# Autodesk Inventor assembly: Sosna
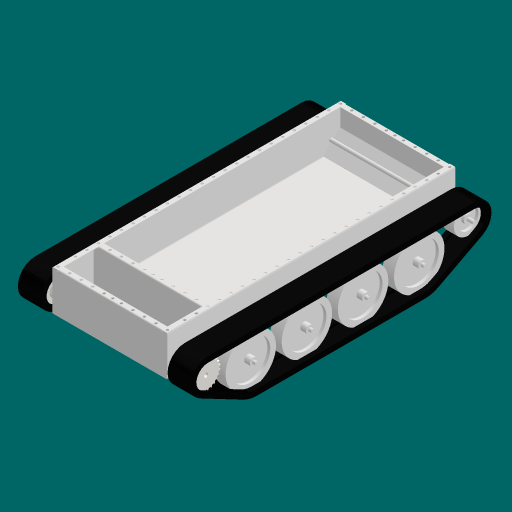
[picture p0: Inventor's stored thumbnail of the model, 512x512]
Saved by Autodesk Inventor 2023 (Build 270158000, 158)
## iProperties
Created: 2023-01-04
Part Number: Sosna
Document SubType Name: Weldment
Designer: HeavyDrewno
Weld Material: Welded Aluminum-6061
Author: HeavyDrewno
## Documents named in this file (16)
- C:\Users\HeavyDrewno\Desktop\Sosna\Sonsna light\Sosna.iam
- C:\Users\HeavyDrewno\Desktop\Sosna\Sonsna light\PK.ipt
- C:\Users\HeavyDrewno\Desktop\Sosna\Sonsna light\Plyta.ipt
- C:\Users\HeavyDrewno\Desktop\Sosna\Sonsna light\KN.ipt
- C:\Users\HeavyDrewno\Desktop\Sosna\Sonsna light\COS\Assembly1\Design Accelerator\Roller Chain Sprocket11.ipt
- C:\Users\HeavyDrewno\Desktop\Sosna\Sonsna light\COS\OS.ipt
- C:\Users\HeavyDrewno\Desktop\Sosna\Sonsna light\KZ.ipt
- C:\Users\HeavyDrewno\Desktop\Sosna\Sonsna light\P_TYŁ.ipt
- C:\Users\HeavyDrewno\Desktop\Sosna\Sonsna light\P_PRZ.ipt
- C:\Users\HeavyDrewno\Desktop\Sosna\Sonsna light\U_OS.ipt
- C:\Users\HeavyDrewno\Desktop\Sosna\Sonsna light\GĄ.ipt
- C:\Users\HeavyDrewno\Desktop\Sosna\Sonsna light\COS\Assembly1\Design Accelerator\Roller Chain Sprocket11_MIR.ipt
- C:\Users\HeavyDrewno\Desktop\Sosna\Sonsna light\KZ_MIR.ipt
- C:\Users\HeavyDrewno\Desktop\Sosna\Sonsna light\PK_MIR.ipt
- C:\Users\HeavyDrewno\Desktop\Sosna\Sonsna light\GĄ_MIR.ipt
- C:\Users\HeavyDrewno\Desktop\Sosna\Sonsna light\G_S.ipt
## Components (32 placed, 15 different names)
1. Plyta:1 — Mate:2, Mate:3, Mate:4, Mate:5, Mate:6, Mate:7, Flush:4, Mate:9, Flush:5, Flush:6, Flush:7, Flush:8, Flush:9, Flush:10, Flush:11, Flush:12, Flush:13, Mate:12, Flush:17, Flush:18
2. KN:1
3. Roller Chain Sprocket1:1 — Mate:5, Mate:6, Flush:15
4. OS:1 — Mate:7, Flush:4, Mate:8
5. KZ:1 — Mate:8, Mate:9, Flush:14
6. P_TYŁ:1 — Flush:5, Flush:6
7. P_PRZ:1 — Flush:7, Flush:8
8. GĄ:1 — Flush:15, Mate:12
9. Roller Chain Sprocket11_MIR:1 — Mate:13
10. KZ_MIR:1 — Flush:16
11. PK_MIR:1 — Flush:16
12. PK_MIR:2
13. PK_MIR:3
14. PK_MIR:4
15. GĄ_MIR:1 — Mate:13
16. G_S:1 — Flush:17, Flush:18
17. U_OS:1 — Flush:9, Flush:10, Flush:11, Flush:12, Mate:10
18. U_OS:2
19. U_OS:3
20. U_OS:4
21. U_OS:5
22. U_OS:6
23. U_OS:7
24. U_OS:8
25. OS:2 — Mate:10, Flush:13, Mate:11
26. OS:3
27. OS:4
28. OS:5
29. PK:1 — Mate:11, Flush:14
30. PK:2
31. PK:3
32. PK:4
## Component patterns: (8 elements, first: U_OS:1), (4 elements, first: OS:2), (4 elements, first: PK:1)
## Relationships (27: Flush 15, Mate 12)
- Mate:2: Plyta:1
- Mate:3: Plyta:1
- Mate:4 (-200 mm): Plyta:1
- Mate:5: Plyta:1 ↔ Roller Chain Sprocket1:1
- Mate:6: Plyta:1 ↔ Roller Chain Sprocket1:1
- Mate:7: Plyta:1 ↔ OS:1
- Flush:4 (-100 mm): Plyta:1 ↔ OS:1
- Mate:8: OS:1 ↔ KZ:1
- Mate:9 (39.5 mm): Plyta:1 ↔ KZ:1
- Flush:5: Plyta:1 ↔ P_TYŁ:1
- Flush:6: Plyta:1 ↔ P_TYŁ:1
- Flush:7: Plyta:1 ↔ P_PRZ:1
- Flush:8: Plyta:1 ↔ P_PRZ:1
- Flush:9: Plyta:1 ↔ U_OS:1
- Flush:10: Plyta:1 ↔ U_OS:1
- Flush:11 (194 mm): Plyta:1 ↔ U_OS:1
- Flush:12 (20 mm): Plyta:1 ↔ U_OS:1
- Mate:10: U_OS:1 ↔ OS:2
- Flush:13 (-100 mm): Plyta:1 ↔ OS:2
- Mate:11: OS:2 ↔ PK:1
- Flush:14 (-10 mm): KZ:1 ↔ PK:1
- Flush:15: Roller Chain Sprocket1:1 ↔ GĄ:1
- Mate:12: Plyta:1 ↔ GĄ:1
- Flush:16 (-10 mm): KZ_MIR:1 ↔ PK_MIR:1
- Mate:13: Roller Chain Sprocket11_MIR:1 ↔ GĄ_MIR:1
- Flush:17: Plyta:1 ↔ G_S:1
- Flush:18: Plyta:1 ↔ G_S:1
